# Autodesk Inventor assembly: Assembly
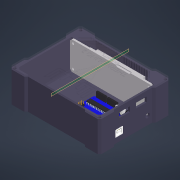
[picture p0: Inventor's stored thumbnail of the model, 180x180]
Saved by Autodesk Inventor 2021.1 (Build 251245010, 245A)
## iProperties
Created: 2020-11-26
Part Number: Assembly
Document SubType Name: Assembly
Designer: Alex
Author: Alex
## Documents named in this file (6)
- C:\Users\Alex\3D Objects\Inventor\Thermolino2_Models\Assembly.iam
- C:\Users\Alex\3D Objects\Inventor\Thermolino2_Models\Case.ipt
- C:\Users\Alex\3D Objects\Inventor\Thermolino2_Models\VFD_Mount.ipt
- C:\Users\Alex\3D Objects\Inventor\Thermolino2_Models\VFD_Dummy.ipt
- C:\Users\Alex\3D Objects\Inventor\Thermolino2_Models\Arduino\arduino uno.iam
- C:\Users\Alex\3D Objects\Inventor\Thermolino2_Models\Lid.ipt
## Components (5 placed, 5 different names)
1. Case:1 — Rotational:3, Rotational:4, Rotational:5, Flush:1, Rotational:8, Rotational:9
2. VFD_Mount:1 — Rotational:3, Rotational:4, Rotational:6, Rotational:7
3. arduino uno:1 [sub-assembly] — Rotational:5
4. VFD_Dummy:1 — Rotational:6, Rotational:7
5. Lid:1 — Rotational:8, Rotational:9
## Relationships (8: RevoluteJoint 7, Flush 1)
- Rotational:3 [RevoluteJoint]: Case:1 ↔ VFD_Mount:1
- Rotational:4 [RevoluteJoint]: Case:1 ↔ VFD_Mount:1
- Rotational:5 [RevoluteJoint]: Case:1 ↔ arduino uno:1
- Rotational:6 [RevoluteJoint]: VFD_Mount:1 ↔ VFD_Dummy:1
- Rotational:7 [RevoluteJoint]: VFD_Mount:1 ↔ VFD_Dummy:1
- Flush:1 (10 mm): Case:1
- Rotational:8 [RevoluteJoint]: Case:1 ↔ Lid:1
- Rotational:9 [RevoluteJoint]: Case:1 ↔ Lid:1
